# Autodesk Inventor assembly: 1x1 Male Header
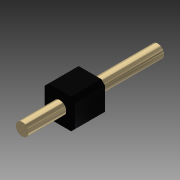
[picture p0: Inventor's stored thumbnail of the model, 180x180]
Saved by Autodesk Inventor 2013 (Build 170138000, 138)
## iProperties
Created: 2014-12-18
Part Number: 1x1 Male Header
Document SubType Name: Assembly
Designer: Kyle
Author: Kyle
## Documents named in this file (3)
- C:\Users\Kyle\Documents\Autodesk\Output\Inventor 2013\Electronics\Headers\Male\1x1 Male Header.iam
- C:\Users\Kyle\Documents\Autodesk\Output\Inventor 2013\Electronics\Sub-Components\Single Bodies\Male Header Base.ipt
- C:\Users\Kyle\Documents\Autodesk\Output\Inventor 2013\Electronics\Sub-Components\Leads\Male Header Lead.ipt
## Components (2 placed, 2 different names)
1. Male Header Base:1 — Mate:1, Flush:1
2. Male Header Lead:1 — Mate:1, Flush:1
## Relationships (2: Mate 1, Flush 1)
- Mate:1: Male Header Base:1 ↔ Male Header Lead:1
- Flush:1 (-3.175 mm): Male Header Base:1 ↔ Male Header Lead:1
